# Autodesk Inventor assembly: am-2492
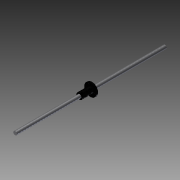
[picture p0: Inventor's stored thumbnail of the model, 180x180]
Saved by Autodesk Inventor 2014 (Build 180170000, 170)
## iProperties
Category: Miscellaneous
Company: Autodesk Inc.
Created: 2013-12-24
Part Number: am-2492
Document SubType Name: Assembly
Designer: Autodesk Inc.
Catalog Web Link: http://www.andymark.com/product-p/am-2492.htm
Vendor: AndyMark
Author: Autodesk Inc.
## Documents named in this file (3)
- D:\Data Folder\FIRST 2014\KOP Parts\Miscellaneous\MISC_LeadScrewAssembly_am-2492.iam
- D:\Data Folder\FIRST 2014\KOP Parts\Miscellaneous\Parts\MISC_LeadScrew_am-2492.ipt
- D:\Data Folder\FIRST 2014\KOP Parts\Miscellaneous\Parts\MISC_LeadNut_am-2492.ipt
## Components (2 placed, 2 different names)
1. MISC_LeadScrew_am-2492:1 — Mate:1
2. MISC_LeadNut_am-2492:1 — Mate:1
## Relationships (1: Mate 1)
- Mate:1: MISC_LeadScrew_am-2492:1 ↔ MISC_LeadNut_am-2492:1
